# Autodesk Inventor assembly: mascon-new
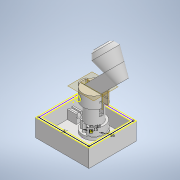
[picture p0: Inventor's stored thumbnail of the model, 180x180]
Saved by Autodesk Inventor 2021 (Build 250183000, 183)
## iProperties
Created: 2021-04-28
Part Number: mascon-new
Document SubType Name: Assembly
Designer: ben
Author: ben
## Documents named in this file (14)
- C:\Users\teh18\OneDrive\BVE Controller\r68-bve-mascon\mascon-new.iam
- C:\Users\teh18\OneDrive\BVE Controller\r68-bve-mascon\mascon.ipt
- C:\Users\teh18\OneDrive\BVE Controller\r68-bve-mascon\handle_base.ipt
- C:\Users\teh18\OneDrive\BVE Controller\r68-bve-mascon\handle_base2.ipt
- C:\Users\teh18\OneDrive\BVE Controller\r68-bve-mascon\stl2\HandleRod1.ipt
- C:\Users\teh18\OneDrive\BVE Controller\r68-bve-mascon\stl2\NotchPiston1.ipt
- C:\Users\teh18\OneDrive\BVE Controller\r68-bve-mascon\stl2\HandleBaseFiller.ipt
- C:\Users\teh18\OneDrive\BVE Controller\r68-bve-mascon\handle-stick.ipt
- C:\Users\teh18\OneDrive\BVE Controller\r68-bve-mascon\handle-sheath.ipt
- C:\Users\teh18\OneDrive\BVE Controller\r68-bve-mascon\stl2\HandleSheathConnector.ipt
- C:\Users\teh18\OneDrive\BVE Controller\r68-bve-mascon\stl2\Handle.iam
- C:\Users\teh18\OneDrive\BVE Controller\potentiometer-b10k-1.snapshot.2\PotentiometerB10K.ipt
- C:\Users\teh18\OneDrive\BVE Controller\r68-bve-mascon\PotHolder.ipt
- C:\Users\teh18\OneDrive\BVE Controller\raspberry-pi-pico-r3-1.snapshot.1\Raspberry Pi Pico-R3.iam
## Components (13 placed, 13 different names)
1. mascon:1 — Flush:3, Mate:3, Mate:4, Tangent:1, Mate:5
2. handle_base:1 — Flush:1, Flush:2, Rotational:1
3. handle_base2:1 — Flush:1
4. HandleRod1:1 — Flush:2
5. NotchPiston1:1 — Flush:3
6. handle-sheath:1 — Mate:1, Mate:2, Flush:4
7. handle-stick:1 — Rotational:1, Mate:1
8. HandleBaseFiller:1
9. HandleSheathConnector:1 — Mate:2, Flush:4
10. Handle:1 [sub-assembly]
11. PotentiometerB10K:1 — Mate:4, Tangent:1
12. PotHolder:1 — Mate:3
13. Raspberry Pi Pico-R3:1 [sub-assembly] — Mate:5
## Relationships (11: Mate 5, Flush 4, RevoluteJoint 1, Tangent 1)
- Flush:1: handle_base:1 ↔ handle_base2:1
- Flush:2: handle_base:1 ↔ HandleRod1:1
- Flush:3: mascon:1 ↔ NotchPiston1:1
- Rotational:1 [RevoluteJoint]: handle_base:1 ↔ handle-stick:1
- Mate:1: handle-sheath:1 ↔ handle-stick:1
- Mate:2: handle-sheath:1 ↔ HandleSheathConnector:1
- Flush:4: handle-sheath:1 ↔ HandleSheathConnector:1
- Mate:3: mascon:1 ↔ PotHolder:1
- Mate:4: mascon:1 ↔ PotentiometerB10K:1
- Tangent:1: mascon:1 ↔ PotentiometerB10K:1
- Mate:5: mascon:1 ↔ Raspberry Pi Pico-R3:1
